# Autodesk Inventor assembly: Assembly5
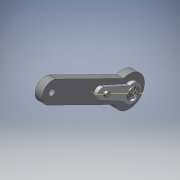
[picture p0: Inventor's stored thumbnail of the model, 180x180]
Saved by Autodesk Inventor 2019.2 (Build 232265000, 265)
## iProperties
Created: 2019-04-09
Part Number: Assembly5
Document SubType Name: Assembly
Designer: richard.girt
Mass: 1.675 g
Surface Area: 15.6 cm^2
Volume: 1.09074 cm^3
Density: 1.53565 g/cm^3
Author: richard.girt
## Documents named in this file (6)
- C:\Users\richard.girt\Desktop\2 Axis robotic arm\Assembly5.iam
- C:\Users\richard.girt\Desktop\2 Axis robotic arm\Part2.ipt
- C:\Users\richard.girt\Desktop\2 Axis robotic arm\SG90Horn1.ipt
- C:\Users\richard.girt\Desktop\2 Axis robotic arm\ANSI B18.6.5M - M2.5x0.45 x 4(38).ipt
- C:\Users\richard.girt\Desktop\2 Axis robotic arm\ANSI B18.6.5M - M2.5x0.45 x 8(38).ipt
- ANSI B18.6.5M - M2.5x0.45 x 8(38).ipt
## Components (4 placed, 4 different names)
1. Part2:1
2. SG90Horn1:1 — Rigid:4
3. ANSI B18.6.5M - M2.5x0.45 x 4(38):1
4. ANSI B18.6.5M - M2.5x0.45 x 8(38):1 — Rigid:4
## Relationships (3: WeldJoint 3)
- [WeldJoint]: SG90Horn1:1 ↔ ANSI B18.6.5M - M2.5x0.45 x 4(38):1
- [WeldJoint]: Part2:1 ↔ SG90Horn1:1
- Rigid:4 [WeldJoint] (-2.8 mm): SG90Horn1:1 ↔ ANSI B18.6.5M - M2.5x0.45 x 8(38):1
